# Autodesk Inventor assembly: SpacingTreads
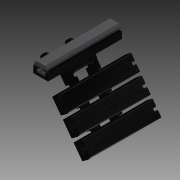
[picture p0: Inventor's stored thumbnail of the model, 180x180]
Saved by Autodesk Inventor 2015 (Build 190159000, 159)
## iProperties
Created: 2015-10-14
Part Number: SpacingTreads
Document SubType Name: Assembly
Designer: nojessen
Author: nojessen
## Documents named in this file (3)
- C:\Users\nojessen\Documents\GitHub\CAD\COTSParts\Tetrix\Tank Treads\SpacingTreads.iam
- C:\Users\nojessen\Documents\GitHub\CAD\COTSParts\Tetrix\Tank Treads\Tank_Tread_without_Rubber.iam
- C:\Users\nojessen\Documents\GitHub\CAD\COTSParts\Tetrix\Tank Treads\Tred Link.iam
## Components (4 placed, 2 different names)
1. Tank_Tread_without_Rubber:1 [sub-assembly] — Mate:1, Flush:1, Flush:3, Mate:3
2. Tank_Tread_without_Rubber:2 [sub-assembly] — Mate:1, Flush:1, Mate:2, Flush:2
3. Tank_Tread_without_Rubber:3 [sub-assembly] — Mate:2, Flush:2
4. Tred Link:1 [sub-assembly] — Flush:3, Mate:3
## Relationships (6: Mate 3, Flush 3)
- Mate:1: Tank_Tread_without_Rubber:1 ↔ Tank_Tread_without_Rubber:2
- Flush:1: Tank_Tread_without_Rubber:1 ↔ Tank_Tread_without_Rubber:2
- Mate:2: Tank_Tread_without_Rubber:2 ↔ Tank_Tread_without_Rubber:3
- Flush:2: Tank_Tread_without_Rubber:2 ↔ Tank_Tread_without_Rubber:3
- Flush:3: Tank_Tread_without_Rubber:1 ↔ Tred Link:1
- Mate:3: Tank_Tread_without_Rubber:1 ↔ Tred Link:1
